# Autodesk Inventor assembly: 02 ASY GBK wall shield 1.1.2
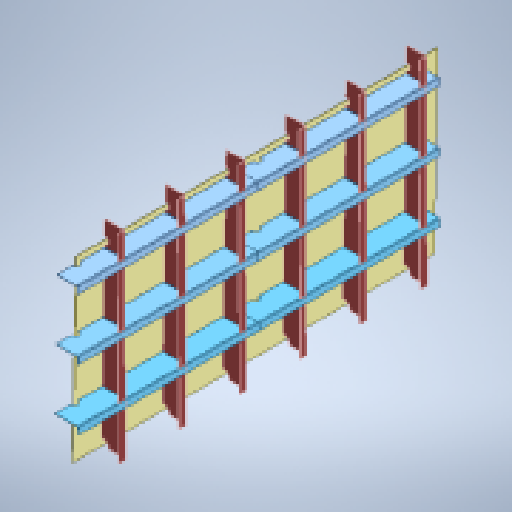
[picture p0: Inventor's stored thumbnail of the model, 512x512]
Saved by Autodesk Inventor 2026.2 (Build 302298000, 298)
## iProperties
Created: 2026-05-07
Part Number: 02 ASY GBK wall shield 1.1.2
Document SubType Name: Assembly
Designer: pokla
Mass: 245734 g
Surface Area: 167509 cm^2
Volume: 31303.7 cm^3
Density: 7.85 g/cm^3
Author: admin
## Documents named in this file (7)
- C:\Users\admin\Documents\Inventor\GBK-Gubkinskiy\02 ASY GBK wall shield 1.1.2.iam
- C:\Users\admin\Documents\Inventor\GBK-Gubkinskiy\0121 GBK shield 2.ipt
- C:\Users\admin\Documents\Inventor\GBK-Gubkinskiy\0234 GBK stringer 1.ipt
- C:\Users\admin\Documents\Inventor\GBK-Gubkinskiy\0235 GBK stringer 2.ipt
- C:\Users\admin\Documents\Inventor\GBK-Gubkinskiy\0236 GBK stringer 3.ipt
- C:\Users\admin\Documents\Inventor\GBK-Gubkinskiy\02.2 GBK rib.ipt
- C:\Users\admin\Documents\Inventor\GBK-Gubkinskiy\01.2 GBK main rib.ipt
## Components (13 placed, 5 different names)
1. 0234 GBK stringer 1:1
2. 0234 GBK stringer 1:2
3. 0235 GBK stringer 2:1
4. 0235 GBK stringer 2:2
5. 0236 GBK stringer 3:1
6. 0236 GBK stringer 3:2
7. 0121 GBK shield 2:1
8. 02.2 GBK rib:1
9. 02.2 GBK rib:2
10. 02.2 GBK rib:3
11. 02.2 GBK rib:4
12. 02.2 GBK rib:5
13. 02.2 GBK rib:6
## Component patterns: (6 elements, first: 02.2 GBK rib:1)
## Relationships (9: WeldJoint 6, Mate 2, Flush 1)
- [WeldJoint]: 0234 GBK stringer 1:1 ↔ 0234 GBK stringer 1:2
- [WeldJoint]: 0235 GBK stringer 2:1 ↔ 0235 GBK stringer 2:2
- [WeldJoint]: 0236 GBK stringer 3:1 ↔ 0236 GBK stringer 3:2
- [Flush] (254 mm): 0121 GBK shield 2:1 ↔ 02.2 GBK rib:1
- [Mate]: 0121 GBK shield 2:1 ↔ 02.2 GBK rib:1
- [Mate]: 0121 GBK shield 2:1 ↔ 02.2 GBK rib:1
- [WeldJoint] (4 mm): 0234 GBK stringer 1:1 ↔ 02.2 GBK rib:1
- [WeldJoint] (4 mm): 0235 GBK stringer 2:1 ↔ 02.2 GBK rib:1
- [WeldJoint] (4 mm): 0236 GBK stringer 3:1 ↔ 02.2 GBK rib:1
## Named parameters: Шаг_шпангоутов = 496.66667 mm
